# Autodesk Inventor assembly: table
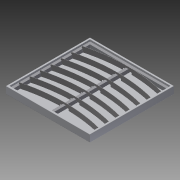
[picture p0: Inventor's stored thumbnail of the model, 180x180]
Saved by Autodesk Inventor 2013 (Build 170138000, 138)
## iProperties
Created: 2012-10-20
Part Number: table
Document SubType Name: Weldment
Designer: Istvan
Weld Material: Welded Aluminum-6061
Mass: 18318.1 g
Surface Area: 68009.8 cm^2
Volume: 8886.11 cm^3
Density: 2.06143 g/cm^3
Author: Istvan
## Documents named in this file (9)
- C:\Users\istvan.burbank\Documents\GitHub\Crown-Fire\CAD\Frame\Table\table.iam
- C:\Users\istvan.burbank\Documents\GitHub\Crown-Fire\CAD\Frame\Table\tableBottom.ipt
- C:\Users\istvan.burbank\Documents\GitHub\Crown-Fire\CAD\Frame\Table\tableSide.ipt
- C:\Users\istvan.burbank\Documents\GitHub\Crown-Fire\CAD\Frame\Table\slats.ipt
- C:\Users\istvan.burbank\Documents\GitHub\Crown-Fire\CAD\Frame\Table\tableFrameLong.ipt
- E:\GitHub\Crown-Fire\CAD\Templates\squareTube1.5x2.ipt
- C:\Users\istvan.burbank\Documents\GitHub\Crown-Fire\CAD\Frame\Table\slatHolder_r.iam
- C:\Users\istvan.burbank\Documents\GitHub\Crown-Fire\CAD\Frame\Table\slatHolder_l.iam
- C:\Users\istvan.burbank\Documents\GitHub\Crown-Fire\CAD\Frame\Table\tableFrameMiddle.ipt
## Components (17 placed, 7 different names)
1. tableBottom:1 — Mate:38, Mate:39, Mate:40, Mate:41, Mate:48, Mate:49, Mate:54, Mate:55, Mate:59, Mate:65, Mate:68, Mate:69
2. tableSide:1 — Mate:40, Mate:44, Mate:45, Mate:46, Mate:47, Mate:49, Mate:51
3. tableSide:2 — Mate:41, Mate:46, Mate:47, Mate:52, Mate:53, Mate:60
4. tableSide:3 — Mate:39, Mate:42, Mate:43, Mate:44, Mate:45, Mate:48, Mate:71
5. tableSide:4 — Mate:38, Mate:42, Mate:43, Mate:50
6. tableFrameLong:1 — Mate:51, Mate:52, Mate:55, Mate:61, Mate:70
7. tableFrameLong:2 — Mate:50, Mate:53, Mate:54, Mate:73
8. slatHolder_r:1 [sub-assembly] — Mate:69, Mate:70, Mate:71, Mate:75
9. slatHolder_l:1 [sub-assembly] — Mate:59, Mate:60, Mate:61, Mate:74
10. tableFrameMiddle:3 — Mate:65, Mate:73, Mate:74, Tangent:1, Mate:76
11. slats:1 — Mate:68, Tangent:1, Mate:75, Mate:76
12. slats:2
13. slats:3
14. slats:4
15. slats:5
16. slats:6
17. slats:7
## Component patterns: (7 elements, first: slats:1)
## Relationships (31: Mate 30, Tangent 1)
- Mate:38: tableBottom:1 ↔ tableSide:4
- Mate:39: tableBottom:1 ↔ tableSide:3
- Mate:40: tableBottom:1 ↔ tableSide:1
- Mate:41: tableBottom:1 ↔ tableSide:2
- Mate:42: tableSide:3 ↔ tableSide:4
- Mate:43: tableSide:3 ↔ tableSide:4
- Mate:44: tableSide:1 ↔ tableSide:3
- Mate:45: tableSide:1 ↔ tableSide:3
- Mate:46: tableSide:1 ↔ tableSide:2
- Mate:47: tableSide:1 ↔ tableSide:2
- Mate:48: tableBottom:1 ↔ tableSide:3
- Mate:49: tableBottom:1 ↔ tableSide:1
- Mate:50: tableSide:4 ↔ tableFrameLong:2
- Mate:51: tableSide:1 ↔ tableFrameLong:1
- Mate:52: tableSide:2 ↔ tableFrameLong:1
- Mate:53: tableSide:2 ↔ tableFrameLong:2
- Mate:54: tableBottom:1 ↔ tableFrameLong:2
- Mate:55: tableBottom:1 ↔ tableFrameLong:1
- Mate:59: tableBottom:1 ↔ slatHolder_l:1
- Mate:60: tableSide:2 ↔ slatHolder_l:1
- Mate:61: tableFrameLong:1 ↔ slatHolder_l:1
- Mate:65: tableBottom:1 ↔ tableFrameMiddle:3
- Mate:68: tableBottom:1 ↔ slats:1
- Mate:69: tableBottom:1 ↔ slatHolder_r:1
- Mate:70: tableFrameLong:1 ↔ slatHolder_r:1
- Mate:71: tableSide:3 ↔ slatHolder_r:1
- Mate:73: tableFrameLong:2 ↔ tableFrameMiddle:3
- Mate:74 (552.45 mm): slatHolder_l:1 ↔ tableFrameMiddle:3
- Tangent:1: tableFrameMiddle:3 ↔ slats:1
- Mate:75: slatHolder_r:1 ↔ slats:1
- Mate:76 (44.45 mm): tableFrameMiddle:3 ↔ slats:1
